# Autodesk Inventor assembly: moving-field-assm
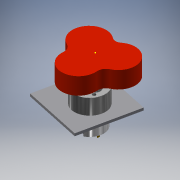
[picture p0: Inventor's stored thumbnail of the model, 180x180]
Saved by Autodesk Inventor 2017 (Build 210142000, 142)
## iProperties
Created: 2017-03-05
Part Number: moving-field-assm
Document SubType Name: Assembly
Designer: John
Author: John
## Documents named in this file (4)
- C:\Users\John\Dropbox\ECE115\pinball-project\moving-field-assm.iam
- C:\Users\John\Dropbox\ECE115\pinball-project\field-mover.ipt
- C:\Users\John\Dropbox\ECE115\geared_DC_Motor.ipt
- C:\Users\John\Dropbox\ECE115\pinball-project\field-mover-motor-case.ipt
## Components (3 placed, 3 different names)
1. field-mover:1 — Mate:1, Mate:2
2. geared_DC_Motor:1 — Mate:1, Mate:2, Mate:3, Mate:4
3. field-mover-motor-case:1 — Mate:3, Mate:4
## Relationships (4: Mate 4)
- Mate:1: field-mover:1 ↔ geared_DC_Motor:1
- Mate:2: field-mover:1 ↔ geared_DC_Motor:1
- Mate:3: geared_DC_Motor:1 ↔ field-mover-motor-case:1
- Mate:4: geared_DC_Motor:1 ↔ field-mover-motor-case:1
